# Autodesk Inventor assembly: 4527 MSFG-24/42-50/60---(0)
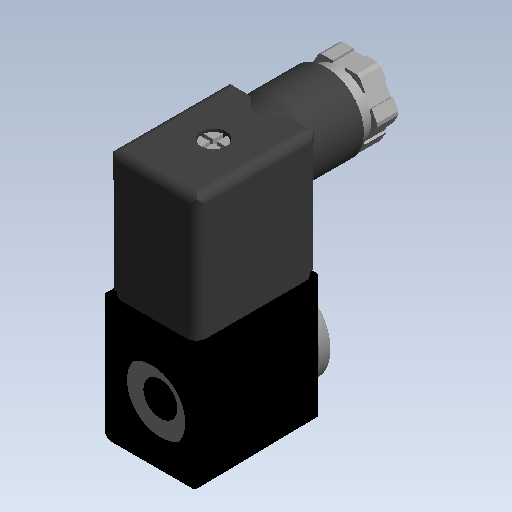
[picture p0: Inventor's stored thumbnail of the model, 512x512]
Saved by Autodesk Inventor 2021 (Build 250183000, 183)
## iProperties
Category: PARTsolutions
Company: FESTO
Part Number: 4527 MSFG-24/42-50/60---(0)
Catalog Web Link: www.cadenas.de
Description: MSFG-Solenoid coil
Vendor: FESTO
Document SubType Name: Assembly
Designer: partserver
Manufacturer: FESTO
Mass: 55 g
Surface Area: 134.6 cm^2
Volume: 38.1773 cm^3
Density: 1.44065 g/cm^3
PSOL_IDENT_0: {ATYP=ASSISTANT},{DATA=script=$CADENAS_DATA/23d-libs/festo/webfesto.vbb/&M_FAMILY=MSFG&M_GROUP=01&M_
PSOL_IDENT_1: PARTNO=4527&IDCODE1=MSFG-24/42-50/60&IDCODE2=&customer_number_cns=&MATES=1&LOD=HI&LOCKERP=0&SINGLEPA
PSOL_IDENT_2: RT=1}
NB: 4527 MSFG-24/42-50/60---(0)
NN: MSFG
NT: Solenoid coil
NBSYN: $TNR. $TYP.---($POS.)
LINA: 4527 MSFG-24/42-50/60---(0)
CATALOG: Festo
TNR: 4527
TYP: MSFG-24/42-50/60
POS: 0
CNSMASSEXACT: 0.055
SUPPLIER: FESTO
ARTICLENO: 4527 MSFG-24/42-50/60---(0)
BOMINFO: 4527 MSFG-24/42-50/60---(0)
CREATOR: CADENAS GmbH
Title: 4527 MSFG-24/42-50/60---(0)
Author: Cadenas PARTsolutions
Comments: Solenoid coil
## Documents named in this file (5)
- C:\Users\Nelson\Github\Proyecto_PAI_2021\01 CAD\Bobina_Electrovalvula.iam
- C:\Users\Nelson\Github\Proyecto_PAI_2021\01 CAD\Bobina_Parte3.ipt
- C:\Users\Nelson\Github\Proyecto_PAI_2021\01 CAD\Bobina_Parte4.ipt
- C:\Users\Nelson\Github\Proyecto_PAI_2021\01 CAD\Bobina_Parte2.ipt
- C:\Users\Nelson\Github\Proyecto_PAI_2021\01 CAD\Bobina_Parte1.ipt
## Components (4 placed, 4 different names)
1. Bobina_Parte3:1 — IP1_XY@1 <-> IP1_XY@2, IP1_Z@1 <-> IP1_Z@2, IP1_YZ@1 <-> IP1_YZ@2, ANBAU_Stecker_XY@1 <-> 2SOC_XY@4, ANBAU_Stecker_Z@1 <-> 2SOC_Z@4, ANBAU_Stecker_YZ@1 <-> 2SOC_YZ@4
2. Bobina_Parte4:1 — IP1_XY@1 <-> IP1_XY@2, IP1_Z@1 <-> IP1_Z@2, IP1_YZ@1 <-> IP1_YZ@2, IP2_XY@2 <-> ANBAU_XY@3, IP2_Z@2 <-> ANBAU_Z@3, IP2_YZ@2 <-> ANBAU_YZ@3
3. Bobina_Parte2:1 — IP2_XY@2 <-> ANBAU_XY@3, IP2_Z@2 <-> ANBAU_Z@3, IP2_YZ@2 <-> ANBAU_YZ@3
4. Bobina_Parte1:1 — ANBAU_Stecker_XY@1 <-> 2SOC_XY@4, ANBAU_Stecker_Z@1 <-> 2SOC_Z@4, ANBAU_Stecker_YZ@1 <-> 2SOC_YZ@4
## Relationships (9: Mate 5, Angle 3, Flush 1)
- IP1_XY@1 <-> IP1_XY@2 [Mate]: Bobina_Parte3:1 ↔ Bobina_Parte4:1
- IP1_Z@1 <-> IP1_Z@2 [Mate]: Bobina_Parte3:1 ↔ Bobina_Parte4:1
- IP1_YZ@1 <-> IP1_YZ@2 [Angle] (0 deg): Bobina_Parte3:1 ↔ Bobina_Parte4:1
- IP2_XY@2 <-> ANBAU_XY@3 [Flush] (0.4 mm): Bobina_Parte4:1 ↔ Bobina_Parte2:1
- IP2_Z@2 <-> ANBAU_Z@3 [Mate]: Bobina_Parte4:1 ↔ Bobina_Parte2:1
- IP2_YZ@2 <-> ANBAU_YZ@3 [Angle] (0 deg): Bobina_Parte4:1 ↔ Bobina_Parte2:1
- ANBAU_Stecker_XY@1 <-> 2SOC_XY@4 [Mate]: Bobina_Parte3:1 ↔ Bobina_Parte1:1
- ANBAU_Stecker_Z@1 <-> 2SOC_Z@4 [Mate]: Bobina_Parte3:1 ↔ Bobina_Parte1:1
- ANBAU_Stecker_YZ@1 <-> 2SOC_YZ@4 [Angle] (0 deg): Bobina_Parte3:1 ↔ Bobina_Parte1:1
